# Autodesk Inventor assembly: 조립품1
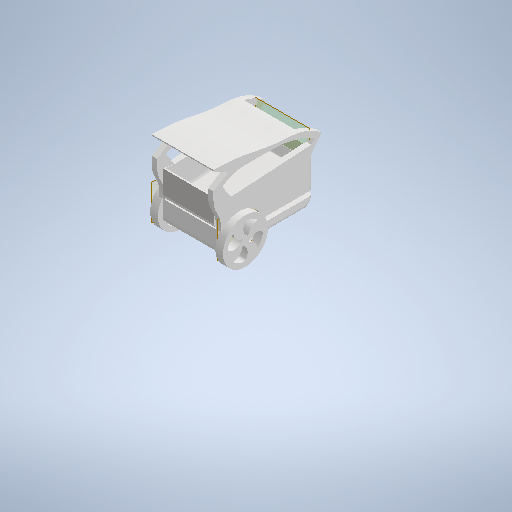
[picture p0: Inventor's stored thumbnail of the model, 512x512]
Saved by Autodesk Inventor 2025 (Build 290162010, 162A)
## iProperties
Created: 2024-05-29
Part Number: 조립품1
Document SubType Name: Assembly
Designer: user
Author: user
## Documents named in this file (7)
- J:\Inventor Files\RoProg24-1\조립품1.iam
- J:\Inventor Files\RoProg24-1\본체 수정.ipt
- J:\Inventor Files\RoProg24-1\바퀴.ipt
- J:\Inventor Files\RoProg24-1\후눈.ipt
- J:\Inventor Files\RoProg24-1\Caster Ball Wheel\Caster Ball Wheel.ipt
- J:\Inventor Files\RoProg24-1\바퀴_반대.ipt
- C:\Users\user\Documents\slider.ipt
## Components (6 placed, 6 different names)
1. 본체 수정:1 — 플러쉬:1, 회전:1, 메이트:2, 회전:3, 회전:4, 슬라이더:1
2. 후눈:1 — 플러쉬:1, 회전:1, 플러쉬:3
3. Caster Ball Wheel:1 — 메이트:2
4. 바퀴:2 — 회전:4
5. 바퀴_반대:1 — 회전:3
6. slider:1 — 플러쉬:3, 슬라이더:1
## Relationships (7: RevoluteJoint 3, Flush 2, Mate 1, TranslationJoint 1)
- 플러쉬:1 [Flush]: 본체 수정:1 ↔ 후눈:1
- 회전:1 [RevoluteJoint]: 본체 수정:1 ↔ 후눈:1
- 메이트:2 [Mate]: 본체 수정:1 ↔ Caster Ball Wheel:1
- 회전:3 [RevoluteJoint]: 본체 수정:1 ↔ 바퀴_반대:1
- 회전:4 [RevoluteJoint]: 본체 수정:1 ↔ 바퀴:2
- 플러쉬:3 [Flush]: 후눈:1 ↔ slider:1
- 슬라이더:1 [TranslationJoint]: 본체 수정:1 ↔ slider:1
